# Autodesk Inventor assembly: Cuerpo
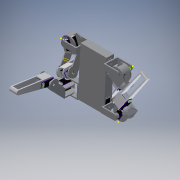
[picture p0: Inventor's stored thumbnail of the model, 180x180]
Saved by Autodesk Inventor 2018 (Build 220112000, 112)
## iProperties
robot-weight-kg: -10.0
robot-prefer-metric: False
robot-driveTrainType: 3
has-driver: False
weight: 10.0
num-sensors: 0
Created: 2020-03-08
Part Number: Cuerpo
Document SubType Name: Assembly
Designer: GonzaloDiaz
Mass: 1251.15 g
Surface Area: 4737 cm^2
Volume: 1216.79 cm^3
Density: 1.02824 g/cm^3
Author: GonzaloDiaz
## Documents named in this file (8)
- E:\Universidad\Codigo\Enigma\Diseños\Cuerpo.iam
- E:\Universidad\Codigo\Enigma\Diseños\Pierna.iam
- E:\Universidad\Codigo\Enigma\Diseños\Pierna_opuesta.iam
- E:\Universidad\Codigo\Enigma\Diseños\Tronco.ipt
- E:\Universidad\Codigo\Enigma\Diseños\SERVOMG996R.ipt
- E:\Universidad\Codigo\Enigma\Diseños\SERVOMG996R_MIR.ipt
- E:\Universidad\Codigo\Enigma\Diseños\SERVOMG996R_MIR1.ipt
- E:\Universidad\Codigo\Enigma\Diseños\SERVOMG996R_MIR_MIR.ipt
## Components (9 placed, 7 different names)
1. Pierna:1 [sub-assembly] — Insert:1, Rotational:1
2. Pierna:2 [sub-assembly] — Insert:3, Rotational:2
3. Pierna_opuesta:1 [sub-assembly] — Insert:2, Rotational:4
4. Pierna_opuesta:2 [sub-assembly] — Insert:4, Rotational:3
5. Tronco:1 — Mate:4, Angle:1, Mate:5, Angle:2, Mate:6, Angle:3, Mate:7, Angle:4, Symmetry:2, Flush:2, Mate:8, Mate:9, Mate:10, Mate:11, Mate:12, Mate:13, Mate:14, Mate:15, Mate:16, Mate:17, Mate:18
6. SERVOMG996R:3 — Mate:8, Mate:9, Mate:10, Insert:2, Rotational:4
7. SERVOMG996R_MIR:1 — Mate:11, Mate:12, Mate:13, Insert:1, Rotational:1
8. SERVOMG996R_MIR1:1 — Mate:16, Mate:17, Mate:18, Insert:4, Rotational:3
9. SERVOMG996R_MIR_MIR:1 — Flush:2, Mate:14, Mate:15, Insert:3, Rotational:2
## Relationships (30: Mate 15, Angle 4, Insert 4, RevoluteJoint 4, Symmetry 2, Flush 1)
- Mate:4: Tronco:1
- Angle:1 (0 deg): Tronco:1
- Mate:5: Tronco:1
- Angle:2 (0 deg): Tronco:1
- Symmetry:1
- Mate:6: Tronco:1
- Angle:3 (0 deg): Tronco:1
- Mate:7: Tronco:1
- Angle:4 (0 deg): Tronco:1
- Symmetry:2: Tronco:1
- Flush:2: Tronco:1 ↔ SERVOMG996R_MIR_MIR:1
- Mate:8: Tronco:1 ↔ SERVOMG996R:3
- Mate:9: Tronco:1 ↔ SERVOMG996R:3
- Mate:10: Tronco:1 ↔ SERVOMG996R:3
- Mate:11: Tronco:1 ↔ SERVOMG996R_MIR:1
- Mate:12: Tronco:1 ↔ SERVOMG996R_MIR:1
- Mate:13: Tronco:1 ↔ SERVOMG996R_MIR:1
- Mate:14: Tronco:1 ↔ SERVOMG996R_MIR_MIR:1
- Mate:15: Tronco:1 ↔ SERVOMG996R_MIR_MIR:1
- Mate:16: Tronco:1 ↔ SERVOMG996R_MIR1:1
- Mate:17: Tronco:1 ↔ SERVOMG996R_MIR1:1
- Mate:18: Tronco:1 ↔ SERVOMG996R_MIR1:1
- Insert:1: Pierna:1 ↔ SERVOMG996R_MIR:1
- Insert:2: Pierna_opuesta:1 ↔ SERVOMG996R:3
- Insert:3: Pierna:2 ↔ SERVOMG996R_MIR_MIR:1
- Insert:4: Pierna_opuesta:2 ↔ SERVOMG996R_MIR1:1
- Rotational:1 [RevoluteJoint]: Pierna:1 ↔ SERVOMG996R_MIR:1
- Rotational:2 [RevoluteJoint]: Pierna:2 ↔ SERVOMG996R_MIR_MIR:1
- Rotational:3 [RevoluteJoint]: Pierna_opuesta:2 ↔ SERVOMG996R_MIR1:1
- Rotational:4 [RevoluteJoint]: Pierna_opuesta:1 ↔ SERVOMG996R:3
